# Autodesk Inventor assembly: caseHw
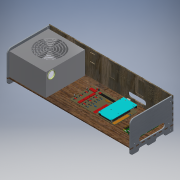
[picture p0: Inventor's stored thumbnail of the model, 180x180]
Saved by Autodesk Inventor 2018.3 (Build 223284000, 284)
## iProperties
Created: 2019-03-04
Part Number: caseHw
Material: Generico
Document SubType Name: Assembly
Designer: AlfyPc
Author: AlfyPc
## Documents named in this file (9)
- C:\Users\AlfyPc\Desktop\Scorbot Hardware\Case Board\caseHw.iam
- C:\Users\AlfyPc\Desktop\Scorbot Hardware\Case Board\LC600H-12.ipt
- C:\Users\AlfyPc\Desktop\Scorbot Hardware\Case Board\tavolaBase.ipt
- C:\Users\AlfyPc\Desktop\Scorbot Hardware\Case Board\Rapsberry\Raspberry Pi 3.iam
- C:\Users\AlfyPc\Desktop\Scorbot Hardware\Case Board\ArduinoMega\ARDUINO MEGA 2560 R3 - Programmable Microcontroller.iam
- C:\Users\AlfyPc\Desktop\Scorbot Hardware\Case Board\moderBoard\matherBoard v1.iam
- C:\Users\AlfyPc\Desktop\Scorbot Hardware\Case Board\LatoAlimentatore.ipt
- C:\Users\AlfyPc\Desktop\Scorbot Hardware\Case Board\Dietro.ipt
- C:\Users\AlfyPc\Desktop\Scorbot Hardware\Case Board\LatoPy.ipt
## Components (8 placed, 8 different names)
1. LC600H-12:1 — Coincidente:1, Coincidente:7, Allineato:3, Allineato:4, Allineato:5
2. tavolaBase:1 — Allineato:1, Coincidente:1, Coincidente:2, Coincidente:6, Allineato:4, Allineato:5, Allineato:6, Allineato:7, Allineato:8
3. Raspberry Pi 3:1 [sub-assembly] — Coincidente:6, Coincidente:8, Allineato:2
4. ARDUINO MEGA 2560 R3 - Programmable Microcontroller:1 [sub-assembly] — Coincidente:3, Coincidente:5, Tangente:1
5. matherBoard v1:1 [sub-assembly] — Coincidente:2, Coincidente:3, Coincidente:5, Tangente:1, Coincidente:7, Coincidente:8, Allineato:2, Allineato:3
6. LatoAlimentatore:1 — Allineato:6
7. Dietro:1 — Allineato:7
8. LatoPy:1 — Allineato:8
## Relationships (16: Flush 8, Mate 7, Tangent 1)
- Allineato:1 [Flush]: tavolaBase:1
- Coincidente:1 [Mate]: LC600H-12:1 ↔ tavolaBase:1
- Coincidente:2 [Mate] (10 mm): tavolaBase:1 ↔ matherBoard v1:1
- Coincidente:3 [Mate]: ARDUINO MEGA 2560 R3 - Programmable Microcontroller:1 ↔ matherBoard v1:1
- Coincidente:5 [Mate] (-14.5 mm): ARDUINO MEGA 2560 R3 - Programmable Microcontroller:1 ↔ matherBoard v1:1
- Coincidente:6 [Mate] (10 mm): tavolaBase:1 ↔ Raspberry Pi 3:1
- Tangente:1: ARDUINO MEGA 2560 R3 - Programmable Microcontroller:1 ↔ matherBoard v1:1
- Coincidente:7 [Mate] (60 mm): LC600H-12:1 ↔ matherBoard v1:1
- Coincidente:8 [Mate] (30 mm): Raspberry Pi 3:1 ↔ matherBoard v1:1
- Allineato:2 [Flush]: Raspberry Pi 3:1 ↔ matherBoard v1:1
- Allineato:3 [Flush] (30 mm): LC600H-12:1 ↔ matherBoard v1:1
- Allineato:4 [Flush] (2.5 mm): LC600H-12:1 ↔ tavolaBase:1
- Allineato:5 [Flush]: LC600H-12:1 ↔ tavolaBase:1
- Allineato:6 [Flush]: tavolaBase:1 ↔ LatoAlimentatore:1
- Allineato:7 [Flush]: tavolaBase:1 ↔ Dietro:1
- Allineato:8 [Flush]: tavolaBase:1 ↔ LatoPy:1
